# Autodesk Inventor assembly: EnsambleSimple
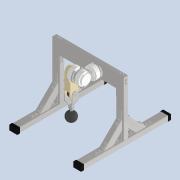
[picture p0: Inventor's stored thumbnail of the model, 180x180]
Saved by Autodesk Inventor 2020.2 (Build 242310000, 310)
## iProperties
Created: 2021-07-23
Part Number: EnsambleSimple
Document SubType Name: Assembly
Designer: Sergio Quintero
Author: Sergio Quintero
## Documents named in this file (5)
- C:\Users\Sergio Quintero\Documents\Universidad\Decimo\PAI\Modelo Simplificado\Piezas simples\EnsambleSimple.iam
- C:\Users\Sergio Quintero\Documents\Universidad\Decimo\PAI\Modelo Simplificado\Piezas simples\Base.ipt
- C:\Users\Sergio Quintero\Documents\Universidad\Decimo\PAI\Modelo Simplificado\Piezas simples\Eslabon1.ipt
- C:\Users\Sergio Quintero\Documents\Universidad\Decimo\PAI\Modelo Simplificado\Piezas simples\Eslabon2.ipt
- C:\Users\Sergio Quintero\Documents\Universidad\Decimo\PAI\Modelo Simplificado\Piezas simples\Eslabon3.ipt
## Components (4 placed, 4 different names)
1. Base:1 — Mate:1, Mate:2
2. Eslabon1:1 — Mate:2, Mate:3
3. Eslabon2:1 — Mate:3, Mate:4
4. Eslabon3:1 — Mate:4
## Relationships (4: Mate 4)
- Mate:1: Base:1
- Mate:2: Base:1 ↔ Eslabon1:1
- Mate:3: Eslabon1:1 ↔ Eslabon2:1
- Mate:4: Eslabon2:1 ↔ Eslabon3:1
